# Autodesk Inventor assembly: GP4-100
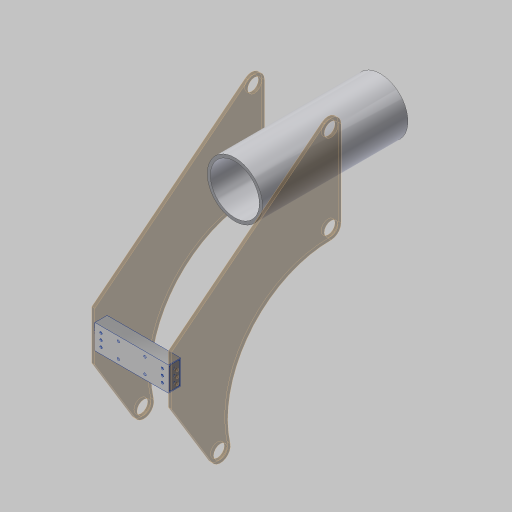
[picture p0: Inventor's stored thumbnail of the model, 512x512]
Saved by Autodesk Inventor 2023.5 (Build 275446000, 446)
## iProperties
Created: 2025-01-28
Part Number: GP4-100
Document SubType Name: Assembly
Designer: slick
Author: slick
## Documents named in this file (6)
- C:\Users\slick\OneDrive\Desktop\2025-ReefScape---CAD\Gripper\GP4\GP4-100.iam
- C:\Users\slick\OneDrive\Desktop\2025-ReefScape---CAD\Gripper\GP4\GP4-001.ipt
- C:\Users\slick\OneDrive\Desktop\2025-ReefScape---CAD\Gripper\GP4\GP4-002.ipt
- C:\Users\slick\OneDrive\Desktop\2025-ReefScape---CAD\Gripper\GP4\GP4-003.ipt
- C:\Users\slick\OneDrive\Desktop\2025-ReefScape---CAD\Gripper\GP4\GP4-003_MIR.ipt
- C:\Users\slick\OneDrive\Desktop\2025-ReefScape---CAD\Field Items\Game Pieces\GE-25500.ipt
## Components (6 placed, 5 different names)
1. GP4-001:1 — Insert:1, Insert:2
2. GP4-002:1 — Flush:1, Flush:2, Flush:3, Mate:1, Flush:4, Flush:5, Angle:1
3. GP4-003:1 — Flush:1, Mate:1, Flush:4, Insert:1, Insert:2
4. GP4-003_MIR:1 — Flush:2, Flush:3, Flush:5, Insert:3, Insert:4
5. GP4-001:2 — Insert:3, Insert:4, Tangent:1, Tangent:2
6. GE-25500:1 — Tangent:1, Tangent:2, Angle:1
## Relationships (13: Flush 5, Insert 4, Tangent 2, Mate 1, Angle 1)
- Flush:1: GP4-002:1 ↔ GP4-003:1
- Flush:2: GP4-002:1 ↔ GP4-003_MIR:1
- Flush:3: GP4-002:1 ↔ GP4-003_MIR:1
- Mate:1: GP4-002:1 ↔ GP4-003:1
- Flush:4: GP4-002:1 ↔ GP4-003:1
- Flush:5: GP4-002:1 ↔ GP4-003_MIR:1
- Insert:1: GP4-001:1 ↔ GP4-003:1
- Insert:2: GP4-001:1 ↔ GP4-003:1
- Insert:3: GP4-003_MIR:1 ↔ GP4-001:2
- Insert:4: GP4-003_MIR:1 ↔ GP4-001:2
- Tangent:1 (19.05 mm): GP4-001:2 ↔ GE-25500:1
- Tangent:2 (19.05 mm): GP4-001:2 ↔ GE-25500:1
- Angle:1 (0 deg): GP4-002:1 ↔ GE-25500:1
